# Autodesk Inventor assembly: Cylinder Slidey Bit
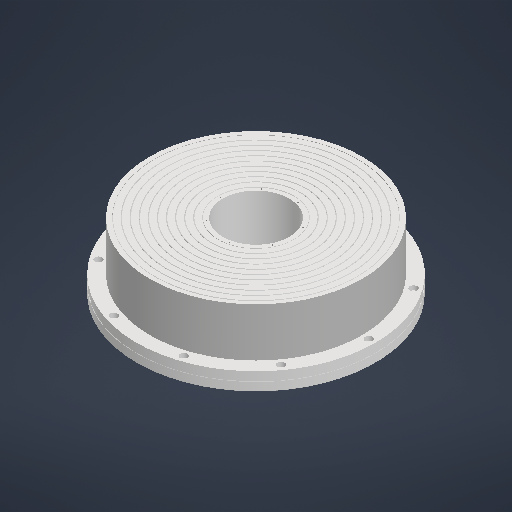
[picture p0: Inventor's stored thumbnail of the model, 512x512]
Saved by Autodesk Inventor 2025 (Build 290162000, 162)
## iProperties
Created: 2024-04-12
Part Number: Cylinder Slidey Bit
Document SubType Name: Assembly
Designer: Thienan Hoang
Author: Thienan Hoang
## Documents named in this file (14)
- C:\Users\mayhe\OneDrive\Documents\GitHub\In-situ-monitoring-of-powder-bed-fusion-additive-manufacturing\system_development\custom-cover\v0.1\hardware design\cylinder-parts\whole-pieces\Cylinder Slidey Bit.iam
- C:\Users\mayhe\OneDrive\Documents\GitHub\In-situ-monitoring-of-powder-bed-fusion-additive-manufacturing\system_development\custom-cover\v0.1\hardware design\cylinder-parts\whole-pieces\Cylinder Slidey Bit Housing.ipt
- C:\Users\mayhe\OneDrive\Documents\GitHub\In-situ-monitoring-of-powder-bed-fusion-additive-manufacturing\system_development\custom-cover\v0.1\hardware design\cylinder-parts\cylinder-segments\Cylinder Segment - 01.ipt
- D:\Research Program thing\Custom Cover\Cylinder\Cylinder Slidey Bit Parts\Cylinder Segments\Cylinder Segment .ipt
- C:\Users\mayhe\OneDrive\Documents\GitHub\In-situ-monitoring-of-powder-bed-fusion-additive-manufacturing\system_development\custom-cover\v0.1\hardware design\cylinder-parts\cylinder-segments\Cylinder Segment - 02.ipt
- C:\Users\mayhe\OneDrive\Documents\GitHub\In-situ-monitoring-of-powder-bed-fusion-additive-manufacturing\system_development\custom-cover\v0.1\hardware design\cylinder-parts\cylinder-segments\Cylinder Segment - 03.ipt
- C:\Users\mayhe\OneDrive\Documents\GitHub\In-situ-monitoring-of-powder-bed-fusion-additive-manufacturing\system_development\custom-cover\v0.1\hardware design\cylinder-parts\cylinder-segments\Cylinder Segment - 04.ipt
- C:\Users\mayhe\OneDrive\Documents\GitHub\In-situ-monitoring-of-powder-bed-fusion-additive-manufacturing\system_development\custom-cover\v0.1\hardware design\cylinder-parts\cylinder-segments\Cylinder Segment - 05.ipt
- C:\Users\mayhe\OneDrive\Documents\GitHub\In-situ-monitoring-of-powder-bed-fusion-additive-manufacturing\system_development\custom-cover\v0.1\hardware design\cylinder-parts\cylinder-segments\Cylinder Segment - 06.ipt
- C:\Users\mayhe\OneDrive\Documents\GitHub\In-situ-monitoring-of-powder-bed-fusion-additive-manufacturing\system_development\custom-cover\v0.1\hardware design\cylinder-parts\cylinder-segments\Cylinder Segment - 07.ipt
- C:\Users\mayhe\OneDrive\Documents\GitHub\In-situ-monitoring-of-powder-bed-fusion-additive-manufacturing\system_development\custom-cover\v0.1\hardware design\cylinder-parts\cylinder-segments\Cylinder Segment - 08.ipt
- C:\Users\mayhe\OneDrive\Documents\GitHub\In-situ-monitoring-of-powder-bed-fusion-additive-manufacturing\system_development\custom-cover\v0.1\hardware design\cylinder-parts\cylinder-segments\Cylinder Segment - 09.ipt
- C:\Users\mayhe\OneDrive\Documents\GitHub\In-situ-monitoring-of-powder-bed-fusion-additive-manufacturing\system_development\custom-cover\v0.1\hardware design\cylinder-parts\cylinder-segments\Cylinder Segment - 10.ipt
- C:\Users\mayhe\OneDrive\Documents\GitHub\In-situ-monitoring-of-powder-bed-fusion-additive-manufacturing\system_development\custom-cover\v0.1\hardware design\cylinder-parts\cylinder-segments\Cylinder Segment - Face.ipt
## Components (12 placed, 12 different names)
1. Cylinder Slidey Bit Housing:1 — Rotational:11, Rotational:13
2. Cylinder Segment - 02:2 — Rotational:2, Rotational:12, Rotational:14
3. Cylinder Segment - 03:3 — Rotational:2, Rotational:3
4. Cylinder Segment - 04:4 — Rotational:3, Rotational:4
5. Cylinder Segment - 05:5 — Rotational:4, Rotational:5
6. Cylinder Segment - 06:6 — Rotational:5, Rotational:6
7. Cylinder Segment - 07:7 — Rotational:6, Rotational:7
8. Cylinder Segment - 08:8 — Rotational:7, Rotational:8
9. Cylinder Segment - 09:9 — Rotational:8, Rotational:9
10. Cylinder Segment - 10:10 — Rotational:9, Rotational:10
11. Cylinder Segment - Face:11 — Rotational:10
12. Cylinder Segment - 01:12 — Rotational:11, Rotational:12, Rotational:13, Rotational:14
## Relationships (13: RevoluteJoint 13)
- Rotational:2 [RevoluteJoint]: Cylinder Segment - 02:2 ↔ Cylinder Segment - 03:3
- Rotational:3 [RevoluteJoint]: Cylinder Segment - 03:3 ↔ Cylinder Segment - 04:4
- Rotational:4 [RevoluteJoint]: Cylinder Segment - 04:4 ↔ Cylinder Segment - 05:5
- Rotational:5 [RevoluteJoint]: Cylinder Segment - 05:5 ↔ Cylinder Segment - 06:6
- Rotational:6 [RevoluteJoint]: Cylinder Segment - 06:6 ↔ Cylinder Segment - 07:7
- Rotational:7 [RevoluteJoint]: Cylinder Segment - 07:7 ↔ Cylinder Segment - 08:8
- Rotational:8 [RevoluteJoint]: Cylinder Segment - 08:8 ↔ Cylinder Segment - 09:9
- Rotational:9 [RevoluteJoint]: Cylinder Segment - 09:9 ↔ Cylinder Segment - 10:10
- Rotational:10 [RevoluteJoint]: Cylinder Segment - 10:10 ↔ Cylinder Segment - Face:11
- Rotational:11 [RevoluteJoint]: Cylinder Slidey Bit Housing:1 ↔ Cylinder Segment - 01:12
- Rotational:12 [RevoluteJoint]: Cylinder Segment - 02:2 ↔ Cylinder Segment - 01:12
- Rotational:13 [RevoluteJoint]: Cylinder Slidey Bit Housing:1 ↔ Cylinder Segment - 01:12
- Rotational:14 [RevoluteJoint]: Cylinder Segment - 02:2 ↔ Cylinder Segment - 01:12
